# Autodesk Inventor assembly: TG-99D
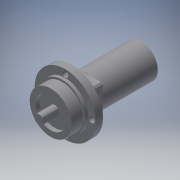
[picture p0: Inventor's stored thumbnail of the model, 180x180]
Saved by Autodesk Inventor 2016 (Build 200138000, 138)
## iProperties
Created: 2016-06-23
Part Number: TG-99D
Material: 一般
Document SubType Name: Assembly
Designer: 宏太
Mass: 227.62 g
Surface Area: 390.94 cm^2
Volume: 227.62 cm^3
Density: 1 g/cm^3
Author: 宏太
## Documents named in this file (5)
- C:\Users\宏太\Documents\Inventor\Content Center Files\Tomoto2016\TukasaMotor\TG-99D.iam
- C:\Users\宏太\Documents\Inventor\Content Center Files\Tomoto2016\TukasaMotor\GearHead1.ipt
- C:\Users\宏太\Documents\Inventor\Content Center Files\Tomoto2016\TukasaMotor\GearHead2.ipt
- C:\Users\宏太\Documents\Inventor\Content Center Files\Tomoto2016\TukasaMotor\motor.ipt
- C:\Users\宏太\Documents\Inventor\Content Center Files\Tomoto2016\TukasaMotor\shaft.ipt
## Components (4 placed, 4 different names)
1. GearHead1:1 — 挿入:1, 挿入:2
2. GearHead2:1 — 挿入:1, 挿入:3
3. motor:1 — 挿入:2
4. shaft:1 — 挿入:3
## Relationships (3: Insert 3)
- 挿入:1 [Insert]: GearHead1:1 ↔ GearHead2:1
- 挿入:2 [Insert]: GearHead1:1 ↔ motor:1
- 挿入:3 [Insert] (-4 mm): GearHead2:1 ↔ shaft:1
